# Autodesk Inventor assembly: 5 Support Model
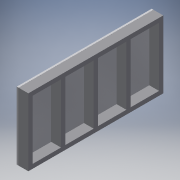
[picture p0: Inventor's stored thumbnail of the model, 180x180]
Saved by Autodesk Inventor 2017 (Build 210142000, 142)
## iProperties
Created: 2017-05-25
Part Number: 5 Support Model
Document SubType Name: Assembly
Designer: cas7
Author: cas7
## Documents named in this file (4)
- C:\Users\Public\Documents\Autodesk\.desktop-connect\.docstore\guided-tutorial-plugin\INVNTOR\5 Support Model.iam
- C:\Users\Public\Documents\Autodesk\.desktop-connect\.docstore\guided-tutorial-plugin\INVNTOR\2017\ENU\552100320579484105\TutorialModelPath\48in 2x4.ipt
- C:\Users\Public\Documents\Autodesk\.desktop-connect\.docstore\guided-tutorial-plugin\INVNTOR\2017\ENU\552100320579484105\TutorialModelPath\21in 2x4.ipt
- C:\Users\Public\Documents\Autodesk\.desktop-connect\.docstore\guided-tutorial-plugin\INVNTOR\2017\ENU\552100320579484105\TutorialModelPath\4x2 Gyp Board.ipt
## Components (8 placed, 2 different names)
1. 4ft 2x4:1 — Mate:13, Mate:14, Mate:15, Mate:16, Mate:17, Mate:18
2. 4ft 2x4:2
3. 4ft 2x4:5 — Mate:19, Mate:24
4. 4ft 2x4:6 — Mate:20, Mate:21, Mate:22, Mate:23, Mate:24
5. 4ft 2x4:7 — Mate:13, Mate:16, Mate:23
6. 4ft 2x4:8 — Mate:14, Mate:17, Mate:21
7. 4ft 2x4:9 — Mate:15, Mate:18, Mate:22
8. 4x2 Gyp Board:1 — Mate:19, Mate:20
## Relationships (19: Mate 19)
- [Mate]: 4ft 2x4:1 ↔ 4ft 2x4:2
- [Mate]: 4ft 2x4:1 ↔ 4ft 2x4:2
- [Mate]: 4ft 2x4:1 ↔ 4ft 2x4:2
- [Mate]: 4ft 2x4:1 ↔ 4ft 2x4:5
- [Mate]: 4ft 2x4:1 ↔ 4ft 2x4:5
- [Mate]: 4ft 2x4:2 ↔ 4ft 2x4:6
- [Mate]: 4ft 2x4:2 ↔ 4ft 2x4:6
- Mate:13: 4ft 2x4:1 ↔ 4ft 2x4:7
- Mate:14: 4ft 2x4:1 ↔ 4ft 2x4:8
- Mate:15: 4ft 2x4:1 ↔ 4ft 2x4:9
- Mate:16: 4ft 2x4:1 ↔ 4ft 2x4:7
- Mate:17: 4ft 2x4:1 ↔ 4ft 2x4:8
- Mate:18: 4ft 2x4:1 ↔ 4ft 2x4:9
- Mate:19: 4ft 2x4:5 ↔ 4x2 Gyp Board:1
- Mate:20: 4ft 2x4:6 ↔ 4x2 Gyp Board:1
- Mate:21: 4ft 2x4:6 ↔ 4ft 2x4:8
- Mate:22: 4ft 2x4:6 ↔ 4ft 2x4:9
- Mate:23: 4ft 2x4:6 ↔ 4ft 2x4:7
- Mate:24: 4ft 2x4:5 ↔ 4ft 2x4:6
